# Autodesk Inventor assembly: SDA 63 50 Full_MIR_MIR
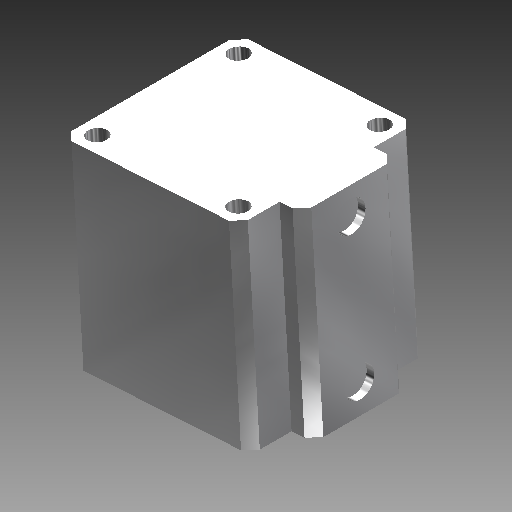
[picture p0: Inventor's stored thumbnail of the model, 512x512]
Saved by Autodesk Inventor 2019 (Build 230136000, 136)
## iProperties
Created: 2019-10-25
Part Number: SDA 63 50 Full_MIR_MIR
Document SubType Name: Assembly
Designer: Mark
Author: Mark
## Documents named in this file (3)
- C:\Users\Mark\Desktop\7738 Helion Engineering\7738-CAD-prep\Butterfly Drive Mk2\Butterfly Base\SDA 63 50 Full_MIR_MIR.iam
- C:\Users\Mark\Desktop\7738 Helion Engineering\7738-CAD-prep\Butterfly drive\SDA 63 50_MIR1_MIR.ipt
- C:\Users\Mark\Desktop\7738 Helion Engineering\7738-CAD-prep\Butterfly drive\SDA 63 50 Stroke Full_MIR1_MIR.ipt
## Components (2 placed, 2 different names)
1. SDA 63 50_MIR1_MIR:1 — Mate:1, Flush:1
2. SDA 63 50 Stroke Full_MIR1_MIR:1 — Mate:1, Flush:1
## Relationships (2: Mate 1, Flush 1)
- Mate:1: SDA 63 50_MIR1_MIR:1 ↔ SDA 63 50 Stroke Full_MIR1_MIR:1
- Flush:1: SDA 63 50_MIR1_MIR:1 ↔ SDA 63 50 Stroke Full_MIR1_MIR:1
